# Autodesk Inventor assembly: Assembly1
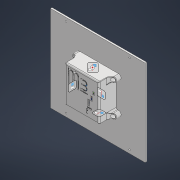
[picture p0: Inventor's stored thumbnail of the model, 180x180]
Saved by Autodesk Inventor 2022 (Build 260153000, 153)
## iProperties
Created: 2021-07-06
Part Number: Assembly1
Document SubType Name: Assembly
Designer: capta
Author: capta
## Documents named in this file (5)
- C:\Users\capta\OneDrive - Lehigh University\Research\Laser-Attenuator-Controller\3d_models\PCB_shield\Assembly1.iam
- C:\Users\capta\OneDrive - Lehigh University\Research\Laser-Attenuator-Controller\3d_models\PCB_shield\shield.ipt
- C:\Users\capta\OneDrive - Lehigh University\Research\Laser-Attenuator-Controller\3d_models\laser_pcb.ipt
- C:\Users\capta\OneDrive - Lehigh University\Research\Laser-Attenuator-Controller\3d_models\side plate.ipt
- C:\Users\capta\OneDrive - Lehigh University\Research\Laser-Attenuator-Controller\3d_models\PCB_shield\Tornillo acero M3x6mm.ipt
## Components (4 placed, 4 different names)
1. shield:1 — Mate:5, Mate:6, Mate:7
2. laser_pcb:1 — Mate:1, Mate:2, Flush:1, Mate:6
3. side plate:1 — Mate:1, Mate:2, Mate:7
4. Tornillo acero M3x6mm:1
## Relationships (6: Mate 5, Flush 1)
- Mate:1 (10 mm): laser_pcb:1 ↔ side plate:1
- Mate:2: laser_pcb:1 ↔ side plate:1
- Flush:1 (-25.379 mm): laser_pcb:1
- Mate:5: shield:1
- Mate:6: shield:1 ↔ laser_pcb:1
- Mate:7: shield:1 ↔ side plate:1
